# Autodesk Inventor assembly: Side Clamping
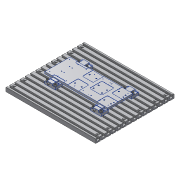
[picture p0: Inventor's stored thumbnail of the model, 180x180]
Saved by Autodesk Inventor 2016 (Build 200138000, 138)
## iProperties
Created: 2015-08-18
Part Number: Side Clamping
Document SubType Name: Assembly
## Documents named in this file (5)
- E:\GitHub\CNC-Router_Z-Axis\Grundplatte_CAM1.iam
- E:\GitHub\CNC-Router\T-Nutenplatte.ipt
- E:\GitHub\CNC-Router_Accessories\Holding Block Assembly.iam
- E:\GitHub\CNC-Router_Accessories\Clamping Block Assembly.iam
- E:\GitHub\CNC-Router_Z-Axis\Grundplatte.ipt
## Components (6 placed, 4 different names)
1. T-Nutenplatte:1 — Mate:1, Mate:3, Mate:7, Mate:12, Mate:13, Mate:16, Flush:4, Flush:5, Mate:18
2. Holding Block Assembly:2 [sub-assembly] — Mate:1, Mate:3, Mate:9, Mate:10, Flush:1, Flush:4
3. Clamping Block Assembly:2 [sub-assembly] — Mate:7, Mate:11, Mate:12, Flush:1, Flush:3, Mate:17
4. Grundplatte:1 — Mate:9, Mate:10, Mate:11, Mate:14, Mate:15, Mate:17
5. Holding Block Assembly:3 [sub-assembly] — Mate:15, Mate:16, Flush:5
6. Clamping Block Assembly:3 [sub-assembly] — Flush:3, Mate:13, Mate:14, Mate:18
## Relationships (18: Mate 13, Flush 5)
- Mate:1: T-Nutenplatte:1 ↔ Holding Block Assembly:2
- Mate:3: T-Nutenplatte:1 ↔ Holding Block Assembly:2
- Mate:7: T-Nutenplatte:1 ↔ Clamping Block Assembly:2
- Mate:9: Holding Block Assembly:2 ↔ Grundplatte:1
- Mate:10: Holding Block Assembly:2 ↔ Grundplatte:1
- Mate:11: Clamping Block Assembly:2 ↔ Grundplatte:1
- Mate:12: T-Nutenplatte:1 ↔ Clamping Block Assembly:2
- Flush:1: Holding Block Assembly:2 ↔ Clamping Block Assembly:2
- [Flush]: Holding Block Assembly:3 ↔ Clamping Block Assembly:3
- Flush:3: Clamping Block Assembly:2 ↔ Clamping Block Assembly:3
- Mate:13: T-Nutenplatte:1 ↔ Clamping Block Assembly:3
- Mate:14: Grundplatte:1 ↔ Clamping Block Assembly:3
- Mate:15: Grundplatte:1 ↔ Holding Block Assembly:3
- Mate:16: T-Nutenplatte:1 ↔ Holding Block Assembly:3
- Flush:4 (80 mm): T-Nutenplatte:1 ↔ Holding Block Assembly:2
- Flush:5 (80 mm): T-Nutenplatte:1 ↔ Holding Block Assembly:3
- Mate:17 (-6 mm): Clamping Block Assembly:2 ↔ Grundplatte:1
- Mate:18: T-Nutenplatte:1 ↔ Clamping Block Assembly:3
## Named parameters: d13_d12 = 0 mm
